# Autodesk Inventor assembly: Rb PEEK
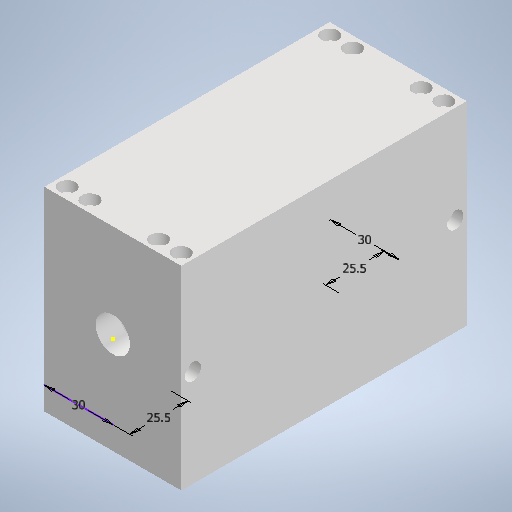
[picture p0: Inventor's stored thumbnail of the model, 512x512]
Saved by Autodesk Inventor 2025.3 (Build 293356000, 356)
## iProperties
Created: 2025-05-09
Part Number: Rb PEEK
Document SubType Name: Assembly
Designer: E. Moreno
Author: E. Moreno
Title: Rb PEEK - Ensamblado
## Documents named in this file (8)
- E:\Users\USER\Documents\GitHub\LAFriOC\Rb oven\Rb PEEK\Rb PEEK.iam
- E:\Users\USER\Documents\GitHub\LAFriOC\Rb oven\Rb PEEK\Rb PEEK - Arriba.ipt
- E:\Users\USER\Documents\GitHub\LAFriOC\Rb oven\Rb PEEK\Rb PEEK - Largo.ipt
- E:\Users\USER\Documents\GitHub\LAFriOC\Rb oven\Rb PEEK\Rb PEEK - Corto con ventana.ipt
- E:\Users\USER\Documents\GitHub\LAFriOC\Rb oven\Rb PEEK\Rb PEEK - Corto.ipt
- E:\Users\USER\Documents\GitHub\LAFriOC\Rb oven\Rb PEEK\Rb PEEK - Largo_MIR.ipt
- E:\Users\USER\Documents\GitHub\LAFriOC\Rb oven\Rb PEEK\Rb PEEK - Arriba_MIR.ipt
- E:\Users\USER\Documents\GitHub\LAFriOC\Rb oven\Rb PEEK\Rb PEEK - Soporte.ipt
## Components (8 placed, 7 different names)
1. Rb PEEK - Arriba:1 — Mate:1, Mate:2, Mate:3, Mate:5, Mate:6, Mate:7, Mate:9, Mate:11, Mate:12
2. Rb PEEK - Largo:1 — Mate:1, Mate:2, Mate:3, Mate:4, Mate:8, Mate:14
3. Rb PEEK - Corto con ventana:1 — Mate:4, Mate:5, Mate:6
4. Rb PEEK - Corto:1 — Mate:7, Mate:8, Mate:9, Mate:10, Mate:13, Mate:15
5. Rb PEEK - Largo_MIR:1 — Mate:10, Mate:11, Mate:12
6. Rb PEEK - Arriba_MIR:1 — Mate:13, Mate:14, Mate:15, Mate:16, Mate:17
7. Rb PEEK - Soporte:1 — Mate:17
8. Rb PEEK - Soporte:2 — Mate:16
## Relationships (17: Mate 17)
- Mate:1: Rb PEEK - Arriba:1 ↔ Rb PEEK - Largo:1
- Mate:2: Rb PEEK - Arriba:1 ↔ Rb PEEK - Largo:1
- Mate:3: Rb PEEK - Arriba:1 ↔ Rb PEEK - Largo:1
- Mate:4: Rb PEEK - Largo:1 ↔ Rb PEEK - Corto con ventana:1
- Mate:5: Rb PEEK - Arriba:1 ↔ Rb PEEK - Corto con ventana:1
- Mate:6: Rb PEEK - Arriba:1 ↔ Rb PEEK - Corto con ventana:1
- Mate:7: Rb PEEK - Arriba:1 ↔ Rb PEEK - Corto:1
- Mate:8: Rb PEEK - Largo:1 ↔ Rb PEEK - Corto:1
- Mate:9: Rb PEEK - Arriba:1 ↔ Rb PEEK - Corto:1
- Mate:10: Rb PEEK - Corto:1 ↔ Rb PEEK - Largo_MIR:1
- Mate:11: Rb PEEK - Arriba:1 ↔ Rb PEEK - Largo_MIR:1
- Mate:12: Rb PEEK - Arriba:1 ↔ Rb PEEK - Largo_MIR:1
- Mate:13: Rb PEEK - Corto:1 ↔ Rb PEEK - Arriba_MIR:1
- Mate:14: Rb PEEK - Largo:1 ↔ Rb PEEK - Arriba_MIR:1
- Mate:15: Rb PEEK - Corto:1 ↔ Rb PEEK - Arriba_MIR:1
- Mate:16: Rb PEEK - Arriba_MIR:1 ↔ Rb PEEK - Soporte:2
- Mate:17: Rb PEEK - Arriba_MIR:1 ↔ Rb PEEK - Soporte:1
